# Autodesk Inventor assembly: IndexingStructure
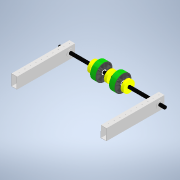
[picture p0: Inventor's stored thumbnail of the model, 180x180]
Saved by Autodesk Inventor 2022 (Build 260153000, 153)
## iProperties
Created: 2022-01-12
Part Number: IndexingStructure
Document SubType Name: Assembly
Designer: merky
Author: merky
## Documents named in this file (6)
- C:\Users\merky\OneDrive\Documents\t3-cad\CAD\2022 Parts\Index\IndexingStructure.iam
- C:\Users\merky\OneDrive\Documents\t3-cad\CAD\2022 Parts\Generic\VersaFrameIndex.ipt
- C:\Users\merky\OneDrive\Documents\t3-cad\CAD\Bearing  for THUNDER.ipt
- C:\Users\merky\OneDrive\Documents\t3-cad\CAD\2022 Parts\Generic\19in thundershaft.ipt
- C:\Users\merky\OneDrive\Documents\t3-cad\CAD\Tristan's CAD\Glock\2 in Compliance Wheel.ipt
- C:\Users\merky\OneDrive\Documents\t3-cad\CAD\2022 Parts\Generic\3in Compliance wheel.ipt
## Components (12 placed, 5 different names)
1. VersaFrameIndex:1 — Flush:1, Flush:2, Insert:2, Insert:5, Mate:1
2. VersaFrameIndex:2 — Flush:1, Flush:2, Insert:4, Insert:7, Mate:1
3. Bearing  for THUNDER:2 — Insert:2
4. Bearing  for THUNDER:3 — Insert:5
5. Bearing  for THUNDER:5 — Insert:7
6. Bearing  for THUNDER:8 — Insert:4, Insert:8
7. 19in thundershaft:1 — Insert:8, Insert:11, Insert:12, Insert:13, Insert:14, Insert:15
8. 2 in Compliance Wheel:1 — Insert:11
9. 2 in Compliance Wheel:2 — Insert:12
10. 2 in Compliance Wheel:3 — Insert:13
11. 3in Compliance wheel:1 — Insert:14
12. 3in Compliance wheel:2 — Insert:15
## Relationships (13: Insert 10, Flush 2, Mate 1)
- Flush:1: VersaFrameIndex:1 ↔ VersaFrameIndex:2
- Flush:2: VersaFrameIndex:1 ↔ VersaFrameIndex:2
- Insert:2: VersaFrameIndex:1 ↔ Bearing  for THUNDER:2
- Insert:4: VersaFrameIndex:2 ↔ Bearing  for THUNDER:8
- Insert:5: VersaFrameIndex:1 ↔ Bearing  for THUNDER:3
- Insert:7: VersaFrameIndex:2 ↔ Bearing  for THUNDER:5
- Mate:1 (381 mm): VersaFrameIndex:1 ↔ VersaFrameIndex:2
- Insert:8 (-457.2 mm): Bearing  for THUNDER:8 ↔ 19in thundershaft:1
- Insert:11 (-254 mm): 19in thundershaft:1 ↔ 2 in Compliance Wheel:1
- Insert:12 (-177.8 mm): 19in thundershaft:1 ↔ 2 in Compliance Wheel:2
- Insert:13 (-330.2 mm): 19in thundershaft:1 ↔ 2 in Compliance Wheel:3
- Insert:14 (-279.4 mm): 19in thundershaft:1 ↔ 3in Compliance wheel:1
- Insert:15 (-218.44 mm): 19in thundershaft:1 ↔ 3in Compliance wheel:2
